# Autodesk Inventor assembly: NCDME075-0600 SMC Pneumatic Cylinder
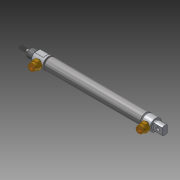
[picture p0: Inventor's stored thumbnail of the model, 180x180]
Saved by Autodesk Inventor 2014 SP1 (Build 180222100, 222)
## iProperties
Created: 2013-12-19
Part Number: NCDME075-0600 SMC Pneumatic Cylinder
Document SubType Name: Assembly
Designer: Moses
Mass: 266.258 g
Surface Area: 438.966 cm^2
Volume: 45.9634 cm^3
Density: 5.79283 g/cm^3
Author: Moses
## Documents named in this file (9)
- C:\Users\Moses\Documents\Inventor\Sally Rebuild\Rebuild Sally\NCDME075-0600 SMC Pneumatic Cylinder.iam
- C:\Users\Moses\Documents\Inventor\Sally Rebuild\Rebuild Sally\Rebuild Shooter NCDME075-0600 Cylinder Front Section.ipt
- C:\Users\Moses\Documents\Inventor\Sally Rebuild\Rebuild Sally\Rebuild Shooter NCDME075-0600 Rod.ipt
- C:\Users\Moses\Documents\Inventor\Sally Rebuild\Rebuild Sally\Rebuild Shooter NCDME075-0600 Body.ipt
- C:\Users\Moses\Documents\Inventor\Sally Rebuild\Rebuild Sally\Pneumatics\Pneumatics_SMC_KQ2H07-34S.ipt
- C:\Users\Moses\Documents\Inventor\Sally Rebuild\Rebuild Sally\Rebuild Shooter NCDME075-0600 Cylinder Bushing.ipt
- C:\Users\Moses\Documents\Inventor\Sally Rebuild\Rebuild Sally\Rebuild Shooter NCDME075-0600 Cylinder Rod Seal.ipt
- C:\Users\Moses\Documents\Inventor\Sally Rebuild\Rebuild Sally\Rebuild Shooter NCDME075-0600 Cylinder Back Section.ipt
- C:\Users\Moses\Documents\Inventor\Sally Rebuild\Rebuild Sally\Rebuild Shooter NCDME075-0600 Piston Seal.ipt
## Components (9 placed, 8 different names)
1. Rebuild Shooter NCDME075-0600 Cylinder Front Section:1 — Flush:3, Mate:1, Mate:3, Tangent:1, Insert:1, Insert:2, Insert:3, Angle:1
2. Rebuild Shooter NCDME075-0600 Rod:1 — Flush:3, Mate:1, Mate:5, Tangent:3
3. Rebuild Shooter NCDME075-0600 Body:1 — Mate:3, Tangent:1, Mate:4, Tangent:2
4. Pneumatics_SMC_KQ2H07-34S:1 — Insert:1
5. Rebuild Shooter NCDME075-0600 Cylinder Bushing:1 — Insert:2
6. Rebuild Shooter NCDME075-0600 Cylinder Rod Seal:1 — Insert:3
7. Rebuild Shooter NCDME075-0600 Cylinder Back Section:1 — Mate:4, Tangent:2, Angle:1, Insert:4
8. Pneumatics_SMC_KQ2H07-34S:2 — Insert:4
9. Rebuild Shooter NCDME075-0600 Piston Seal:1 — Mate:5, Tangent:3
## Relationships (13: Mate 4, Insert 4, Tangent 3, Flush 1, Angle 1)
- Flush:3 (19.05 mm): Rebuild Shooter NCDME075-0600 Cylinder Front Section:1 ↔ Rebuild Shooter NCDME075-0600 Rod:1
- Mate:1: Rebuild Shooter NCDME075-0600 Cylinder Front Section:1 ↔ Rebuild Shooter NCDME075-0600 Rod:1
- Mate:3: Rebuild Shooter NCDME075-0600 Cylinder Front Section:1 ↔ Rebuild Shooter NCDME075-0600 Body:1
- Tangent:1: Rebuild Shooter NCDME075-0600 Cylinder Front Section:1 ↔ Rebuild Shooter NCDME075-0600 Body:1
- Insert:1 (2.54 mm): Rebuild Shooter NCDME075-0600 Cylinder Front Section:1 ↔ Pneumatics_SMC_KQ2H07-34S:1
- Insert:2: Rebuild Shooter NCDME075-0600 Cylinder Front Section:1 ↔ Rebuild Shooter NCDME075-0600 Cylinder Bushing:1
- Insert:3: Rebuild Shooter NCDME075-0600 Cylinder Front Section:1 ↔ Rebuild Shooter NCDME075-0600 Cylinder Rod Seal:1
- Mate:4: Rebuild Shooter NCDME075-0600 Body:1 ↔ Rebuild Shooter NCDME075-0600 Cylinder Back Section:1
- Tangent:2: Rebuild Shooter NCDME075-0600 Body:1 ↔ Rebuild Shooter NCDME075-0600 Cylinder Back Section:1
- Angle:1 (0 deg): Rebuild Shooter NCDME075-0600 Cylinder Front Section:1 ↔ Rebuild Shooter NCDME075-0600 Cylinder Back Section:1
- Insert:4 (2.54 mm): Rebuild Shooter NCDME075-0600 Cylinder Back Section:1 ↔ Pneumatics_SMC_KQ2H07-34S:2
- Mate:5: Rebuild Shooter NCDME075-0600 Rod:1 ↔ Rebuild Shooter NCDME075-0600 Piston Seal:1
- Tangent:3: Rebuild Shooter NCDME075-0600 Rod:1 ↔ Rebuild Shooter NCDME075-0600 Piston Seal:1
